# Autodesk Inventor assembly: skellett
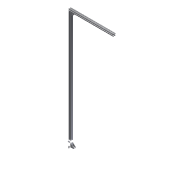
[picture p0: Inventor's stored thumbnail of the model, 180x180]
Saved by Autodesk Inventor 2014 SP1 (Build 180222100, 222)
## iProperties
Created: 2015-02-04
Part Number: skellett
Document SubType Name: Assembly
Designer: Simen
Author: Simen
## Documents named in this file (4)
- C:\Users\Simen\Documents\git\Eit\skjellet\skellett.iam
- C:\Users\Simen\Documents\git\Eit\skjellet\KHFS5_2020_1000.ipt
- C:\Users\Simen\Documents\git\Eit\skjellet\KHFS5_2020_400.ipt
- C:\Users\Simen\Documents\git\Eit\skjellet\jorneFester.iam
## Components (8 placed, 4 different names)
1. KHFS5-2020-400:1 — Flush:4, Mate:2, Mate:3, Flush:7, Flush:8, Flush:9, Mate:5, Mate:6
2. KHFS5-2020-1000:1 — Flush:4, Mate:1, Flush:6, Mate:5, Mate:6
3. jorneFester:1 [sub-assembly] — Mate:1, Flush:6, Mate:2
4. jorneFester:2 [sub-assembly] — Mate:3, Flush:7, Flush:8, Mate:4, Flush:10
5. jorneFester:3 [sub-assembly]
6. jorneFester:4 [sub-assembly]
7. jorneFester:5 [sub-assembly]
8. KHFS5-2020-4000:3 — Mate:4, Flush:9, Flush:10
## Relationships (12: Flush 6, Mate 6)
- Flush:4: KHFS5-2020-400:1 ↔ KHFS5-2020-1000:1
- Mate:1: KHFS5-2020-1000:1 ↔ jorneFester:1
- Flush:6: KHFS5-2020-1000:1 ↔ jorneFester:1
- Mate:2: KHFS5-2020-400:1 ↔ jorneFester:1
- Mate:3: KHFS5-2020-400:1 ↔ jorneFester:2
- Flush:7: KHFS5-2020-400:1 ↔ jorneFester:2
- Flush:8: KHFS5-2020-400:1 ↔ jorneFester:2
- Mate:4: jorneFester:2 ↔ KHFS5-2020-4000:3
- Flush:9: KHFS5-2020-400:1 ↔ KHFS5-2020-4000:3
- Flush:10: jorneFester:2 ↔ KHFS5-2020-4000:3
- Mate:5: KHFS5-2020-400:1 ↔ KHFS5-2020-1000:1
- Mate:6: KHFS5-2020-400:1 ↔ KHFS5-2020-1000:1
